# Autodesk Inventor assembly: back_plates
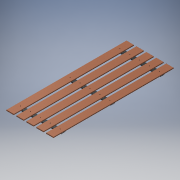
[picture p0: Inventor's stored thumbnail of the model, 180x180]
Saved by Autodesk Inventor 2019 (Build 230136000, 136)
## iProperties
Created: 2019-02-23
Part Number: back_plates
Document SubType Name: Assembly
Designer: gaincarlo
Author: gaincarlo
## Documents named in this file (3)
- D:\Giancarlo Bacchio\Documenti\00 - Progetti\30-Inventor\LaPanca\back_plates.iam
- D:\Giancarlo Bacchio\Documenti\00 - Progetti\30-Inventor\LaPanca\support1.ipt
- D:\Giancarlo Bacchio\Documenti\00 - Progetti\30-Inventor\LaPanca\doga_long1.ipt
## Components (8 placed, 2 different names)
1. support1:1 — Mate:1, Mate:2, Mate:7
2. support1:2 — Mate:3, Mate:5, Mate:9
3. support1:3 — Mate:4, Mate:6, Mate:8
4. doga_long1:1 — Mate:1, Mate:2, Mate:3, Mate:4, Mate:5, Mate:6
5. doga_long1:2
6. doga_long1:3 — Mate:7, Mate:8, Mate:9
7. doga_long1:4
8. doga_long1:5
## Component patterns: (5 elements, first: doga_long1:1)
## Relationships (9: Mate 9)
- Mate:1: support1:1 ↔ doga_long1:1
- Mate:2: support1:1 ↔ doga_long1:1
- Mate:3: support1:2 ↔ doga_long1:1
- Mate:4: support1:3 ↔ doga_long1:1
- Mate:5: support1:2 ↔ doga_long1:1
- Mate:6: support1:3 ↔ doga_long1:1
- Mate:7: support1:1 ↔ doga_long1:3
- Mate:8: support1:3 ↔ doga_long1:3
- Mate:9: support1:2 ↔ doga_long1:3
